# Autodesk Inventor assembly: Traveler Assya
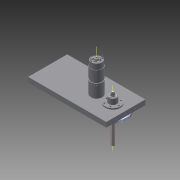
[picture p0: Inventor's stored thumbnail of the model, 180x180]
Saved by Autodesk Inventor 2014 (Build 180170000, 170)
## iProperties
Created: 2015-01-23
Part Number: Traveler Assya
Document SubType Name: Assembly
Designer: chappelled
Author: chappelled
## Documents named in this file (16)
- C:\Users\chappelled\Documents\Inventor\Claw\Traveler Assya.iam
- C:\Users\chappelled\Documents\Inventor\Claw\Traveler.ipt
- C:\Users\chappelled\Documents\Inventor\Claw\.875 Bearing Hub.ipt
- C:\Users\chappelled\Documents\Inventor\Claw\Imported Components\PG-71-am-0914\PG-71-am-0914.ipt
- C:\Users\chappelled\Documents\Inventor\Claw\DBK_FR6ZZBearing_am-0028.ipt
- C:\Users\chappelled\Documents\Inventor\Claw\Imported Components\am-0396+TB+Hex+Long+Output+Shaft\am-0396+TB+Hex+Long+Output+Shaft.ipt
- C:\Users\chappelled\Documents\Inventor\Claw\Imported Components\217-3577-STEP\217-3577-STEP.ipt
- C:\Users\chappelled\Documents\Inventor\Claw\Imported Components\FR8ZZ Hex Bearing.ipt\FR8ZZ Hex Bearing.ipt.ipt
- C:\Users\chappelled\Documents\Inventor\Claw\Imported Components\16T-10mmKeyBoreAM-2088\16T-10mmKeyBoreAM-2088.ipt
- C:\Users\chappelled\Documents\Inventor\Claw\4mm Key.ipt
- C:\Users\chappelled\Documents\Inventor\Content Center Files\R2014\en-US\ASME B18.21.1(02)\ASME B18.21.1 - 1_4 Extra-Duty. Lock Washers (Inch Series)Extra-Duty Helical Spring Lock Washer(7).ipt
- C:\Users\chappelled\Documents\Inventor\Content Center Files\R2014\en-US\IFI 100 107(2)\IFI 100_107 - 1_4 - 20 Metal Type.ipt
- C:\Users\chappelled\Documents\Inventor\Content Center Files\R2014\en-US\ANSI B27.7M\ANSI B27.7M - 3CMI-15.ipt
- C:\Users\chappelled\Documents\Inventor\Claw\Traveler Assy\Design Accelerator\Bolted Connection4.iam
- C:\Users\chappelled\Documents\Inventor\Claw\Traveler Assy\Design Accelerator\Bolted Connection6.iam
- FR8ZZ Hex Bearing.ipt
## Components (14 placed, 13 different names)
1. Traveler:1 — Mate:2, Mate:3, Mate:8, Mate:9, Mate:31, Mate:32, Mate:44, Mate:45, Mate:46, Mate:47
2. .875 Bearing Hub:1 — Mate:2, Mate:3, Mate:9, Mate:16, Mate:17
3. PG-71-am-0914:1 — Mate:8, Mate:26, Mate:27, Flush:1, Mate:29
4. DBK_FR6ZZBearing_am-0028:1 — Mate:16, Mate:17, Mate:18, Mate:19
5. am-0396+TB+Hex+Long+Output+Shaft:1 — Mate:18, Mate:19, Mate:23, Mate:24, Mate:34, Mate:36, Mate:37, Mate:38, Mate:40, Mate:41
6. 217-3577-STEP:1 — Mate:23, Mate:24
7. FR8ZZ Hex Bearing.ipt:1 — Mate:32, Mate:33
8. 16T-10mmKeyBoreAM-2088:1 — Mate:28
9. 4mm Key:2 — Mate:26, Mate:27, Flush:1
10. Extra-Duty Helical Spring Lock Washer (Inch) 1/4 Extra-Duty. Lock Washers (Inch Series)Extra-Duty Helical Spring Lock Washer:1 — Mate:36, Mate:37, Mate:39
11. Prevailing Torque Type Hex Nut - Inch (IFI) 1/4 - 20 Metal Type:1 — Mate:38, Mate:39
12. ANSI B27.7M 3CMI-15:1 — Mate:40, Mate:41
13. Bolted Connection:1 [sub-assembly] — Mate:46, Mate:47
14. Bolted Connection:2 [sub-assembly] — Mate:44, Mate:45
## Relationships (31: Mate 30, Flush 1)
- Mate:2: Traveler:1 ↔ .875 Bearing Hub:1
- Mate:3: Traveler:1 ↔ .875 Bearing Hub:1
- Mate:8: Traveler:1 ↔ PG-71-am-0914:1
- Mate:9: Traveler:1 ↔ .875 Bearing Hub:1
- Mate:16: .875 Bearing Hub:1 ↔ DBK_FR6ZZBearing_am-0028:1
- Mate:17: .875 Bearing Hub:1 ↔ DBK_FR6ZZBearing_am-0028:1
- Mate:18: DBK_FR6ZZBearing_am-0028:1 ↔ am-0396+TB+Hex+Long+Output+Shaft:1
- Mate:19: DBK_FR6ZZBearing_am-0028:1 ↔ am-0396+TB+Hex+Long+Output+Shaft:1
- Mate:23: am-0396+TB+Hex+Long+Output+Shaft:1 ↔ 217-3577-STEP:1
- Mate:24: am-0396+TB+Hex+Long+Output+Shaft:1 ↔ 217-3577-STEP:1
- Mate:26: PG-71-am-0914:1 ↔ 4mm Key:2
- Mate:27: PG-71-am-0914:1 ↔ 4mm Key:2
- Flush:1: PG-71-am-0914:1 ↔ 4mm Key:2
- Mate:28: 16T-10mmKeyBoreAM-2088:1
- Mate:29: PG-71-am-0914:1
- Mate:30
- Mate:31: Traveler:1
- Mate:32: Traveler:1 ↔ FR8ZZ Hex Bearing.ipt:1
- Mate:33: FR8ZZ Hex Bearing.ipt:1
- Mate:34: am-0396+TB+Hex+Long+Output+Shaft:1
- Mate:35
- Mate:36: am-0396+TB+Hex+Long+Output+Shaft:1 ↔ Extra-Duty Helical Spring Lock Washer (Inch) 1/4 Extra-Duty. Lock Washers (Inch Series)Extra-Duty Helical Spring Lock Washer:1
- Mate:37: am-0396+TB+Hex+Long+Output+Shaft:1 ↔ Extra-Duty Helical Spring Lock Washer (Inch) 1/4 Extra-Duty. Lock Washers (Inch Series)Extra-Duty Helical Spring Lock Washer:1
- Mate:38: am-0396+TB+Hex+Long+Output+Shaft:1 ↔ Prevailing Torque Type Hex Nut - Inch (IFI) 1/4 - 20 Metal Type:1
- Mate:39: Extra-Duty Helical Spring Lock Washer (Inch) 1/4 Extra-Duty. Lock Washers (Inch Series)Extra-Duty Helical Spring Lock Washer:1 ↔ Prevailing Torque Type Hex Nut - Inch (IFI) 1/4 - 20 Metal Type:1
- Mate:40: am-0396+TB+Hex+Long+Output+Shaft:1 ↔ ANSI B27.7M 3CMI-15:1
- Mate:41: am-0396+TB+Hex+Long+Output+Shaft:1 ↔ ANSI B27.7M 3CMI-15:1
- Mate:44: Traveler:1 ↔ Bolted Connection:2
- Mate:45: Traveler:1 ↔ Bolted Connection:2
- Mate:46: Traveler:1 ↔ Bolted Connection:1
- Mate:47: Traveler:1 ↔ Bolted Connection:1
